# Autodesk Inventor assembly: __assembly
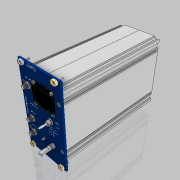
[picture p0: Inventor's stored thumbnail of the model, 180x180]
Saved by Autodesk Inventor 2021.4 (Build 254397000, 397)
## iProperties
Created: 2023-11-08
Part Number: __assembly
Document SubType Name: Assembly
Designer: Tilman Preuschoff
Author: Tilman Preuschoff
## Documents named in this file (12)
- C:\Users\Tilman Preuschoff\Documents\GitHub\PDH-module\frontpanel\assembly\__assembly.iam
- C:\Users\Tilman Preuschoff\Documents\GitHub\PDH-module\frontpanel\assembly\Fischer HB.ipt
- C:\Users\Tilman Preuschoff\Documents\GitHub\PDH-module\frontpanel\assembly\PDH_module.iam
- C:\Users\Tilman Preuschoff\Documents\GitHub\PDH-module\frontpanel\Fischer_TFP.ipt
- C:\Users\Tilman Preuschoff\Documents\GitHub\PDH-module\frontpanel\assembly\display.ipt
- C:\Users\Tilman Preuschoff\Documents\GitHub\PDH-module\frontpanel\assembly\KY-040 Rotary Encoder.ipt
- C:\Users\Tilman Preuschoff\Documents\GitHub\PDH-module\frontpanel\assembly\5230_-_5000_-_panel.iam
- C:\Users\Tilman Preuschoff\Documents\GitHub\PDH-module\frontpanel\assembly\9533ncdk_-_9100-9200-9500.iam
- C:\Users\Tilman Preuschoff\Documents\Inventor\Content Center Files\R2021\de-DE\BS EN ISO 7046-2 H\BS EN ISO 7046-2 H - M3x10 - 8.8 - H1.ipt
- C:\Users\Tilman Preuschoff\Documents\Inventor\Content Center Files\R2021\de-DE\ISO 1207(1)\DIN EN ISO 1207 - M2,5 x 6.ipt
- C:\Users\Tilman Preuschoff\Documents\GitHub\PDH-module\frontpanel\assembly\KN1.ipt
- C:\Users\Tilman Preuschoff\Documents\Inventor\Content Center Files\R2021\de-DE\DIN 7985 (H)\DIN 7985 (H) - M2,5x10-H.ipt
## Components (24 placed, 11 different names)
1. Fischer HB:1 — Passend:1, Passend:2, Passend:3, Passend:4, Fluchtend:1, Fluchtend:2, Passend:5, Fluchtend:3, Passend:6, Passend:7, Passend:8, Passend:9, Passend:10
2. Fischer HB:2 — Fluchtend:1, Fluchtend:2, Passend:5
3. PDH_module:1 [sub-assembly] — Fluchtend:3, Passend:6, Passend:7
4. Fischer_TFP:1 — Passend:8, Passend:9, Passend:10, Passend:11, Passend:12, Passend:13, Passend:14, Passend:15, Passend:16, Passend:17, Starr:1, Drehbar:1, Drehbar:2, Drehbar:3, Drehbar:4, Drehbar:9, Drehbar:10, Drehbar:11, Drehbar:12
5. display:1 — Passend:11, Passend:12, Passend:13, Drehbar:5, Drehbar:6, Drehbar:7, Drehbar:8
6. KY-040 Rotary Encoder:1 — Passend:14, Passend:15
7. 5230_-_5000_-_panel:1 [sub-assembly] — Passend:16, Passend:17
8. 9533ncdk_-_9100-9200-9500:1 [sub-assembly] — Starr:1
9. BS EN ISO 7046-2 H M3x10 - 8.8 - H1:1 — Drehbar:1
10. BS EN ISO 7046-2 H M3x10 - 8.8 - H1:2 — Drehbar:3
11. BS EN ISO 7046-2 H M3x10 - 8.8 - H1:3 — Drehbar:2
12. BS EN ISO 7046-2 H M3x10 - 8.8 - H1:4 — Drehbar:4
13. DIN EN ISO 1207 M2,5 x 6:1 — Drehbar:5
14. DIN EN ISO 1207 M2,5 x 6:2 — Drehbar:6
15. DIN EN ISO 1207 M2,5 x 6:3 — Drehbar:7
16. DIN EN ISO 1207 M2,5 x 6:4 — Drehbar:8
17. KN1:1 — Drehbar:9, Drehbar:13
18. KN1:2 — Drehbar:10, Drehbar:14
19. KN1:3 — Drehbar:11, Drehbar:15
20. KN1:4 — Drehbar:12, Drehbar:16
21. DIN 7985 (H) M2,5x10-H:1 — Drehbar:13
22. DIN 7985 (H) M2,5x10-H:2 — Drehbar:14
23. DIN 7985 (H) M2,5x10-H:3 — Drehbar:15
24. DIN 7985 (H) M2,5x10-H:4 — Drehbar:16
## Relationships (37: Mate 17, RevoluteJoint 16, Flush 3, WeldJoint 1)
- Passend:1 [Mate]: Fischer HB:1
- Passend:2 [Mate]: Fischer HB:1
- Passend:3 [Mate]: Fischer HB:1
- Passend:4 [Mate]: Fischer HB:1
- Fluchtend:1 [Flush]: Fischer HB:1 ↔ Fischer HB:2
- Fluchtend:2 [Flush]: Fischer HB:1 ↔ Fischer HB:2
- Passend:5 [Mate]: Fischer HB:1 ↔ Fischer HB:2
- Fluchtend:3 [Flush]: Fischer HB:1 ↔ PDH_module:1
- Passend:6 [Mate]: Fischer HB:1 ↔ PDH_module:1
- Passend:7 [Mate] (0.2 mm): Fischer HB:1 ↔ PDH_module:1
- Passend:8 [Mate]: Fischer HB:1 ↔ Fischer_TFP:1
- Passend:9 [Mate]: Fischer HB:1 ↔ Fischer_TFP:1
- Passend:10 [Mate]: Fischer HB:1 ↔ Fischer_TFP:1
- Passend:11 [Mate]: Fischer_TFP:1 ↔ display:1
- Passend:12 [Mate]: Fischer_TFP:1 ↔ display:1
- Passend:13 [Mate]: Fischer_TFP:1 ↔ display:1
- Passend:14 [Mate]: Fischer_TFP:1 ↔ KY-040 Rotary Encoder:1
- Passend:15 [Mate]: Fischer_TFP:1 ↔ KY-040 Rotary Encoder:1
- Passend:16 [Mate]: Fischer_TFP:1 ↔ 5230_-_5000_-_panel:1
- Passend:17 [Mate]: Fischer_TFP:1 ↔ 5230_-_5000_-_panel:1
- Starr:1 [WeldJoint] (2.5 mm): Fischer_TFP:1 ↔ 9533ncdk_-_9100-9200-9500:1
- Drehbar:1 [RevoluteJoint]: Fischer_TFP:1 ↔ BS EN ISO 7046-2 H M3x10 - 8.8 - H1:1
- Drehbar:2 [RevoluteJoint]: Fischer_TFP:1 ↔ BS EN ISO 7046-2 H M3x10 - 8.8 - H1:3
- Drehbar:3 [RevoluteJoint]: Fischer_TFP:1 ↔ BS EN ISO 7046-2 H M3x10 - 8.8 - H1:2
- Drehbar:4 [RevoluteJoint]: Fischer_TFP:1 ↔ BS EN ISO 7046-2 H M3x10 - 8.8 - H1:4
- Drehbar:5 [RevoluteJoint]: display:1 ↔ DIN EN ISO 1207 M2,5 x 6:1
- Drehbar:6 [RevoluteJoint]: display:1 ↔ DIN EN ISO 1207 M2,5 x 6:2
- Drehbar:7 [RevoluteJoint]: display:1 ↔ DIN EN ISO 1207 M2,5 x 6:3
- Drehbar:8 [RevoluteJoint]: display:1 ↔ DIN EN ISO 1207 M2,5 x 6:4
- Drehbar:9 [RevoluteJoint]: Fischer_TFP:1 ↔ KN1:1
- Drehbar:10 [RevoluteJoint]: Fischer_TFP:1 ↔ KN1:2
- Drehbar:11 [RevoluteJoint]: Fischer_TFP:1 ↔ KN1:3
- Drehbar:12 [RevoluteJoint]: Fischer_TFP:1 ↔ KN1:4
- Drehbar:13 [RevoluteJoint]: KN1:1 ↔ DIN 7985 (H) M2,5x10-H:1
- Drehbar:14 [RevoluteJoint]: KN1:2 ↔ DIN 7985 (H) M2,5x10-H:2
- Drehbar:15 [RevoluteJoint]: KN1:3 ↔ DIN 7985 (H) M2,5x10-H:3
- Drehbar:16 [RevoluteJoint]: KN1:4 ↔ DIN 7985 (H) M2,5x10-H:4
